# Autodesk Inventor assembly: Flap
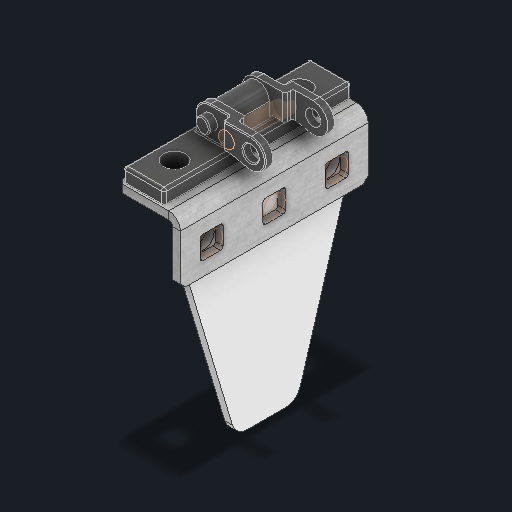
[picture p0: Inventor's stored thumbnail of the model, 512x512]
Saved by Autodesk Inventor 2025.1 (Build 291241000, 241)
## iProperties
Created: 2024-11-18
Part Number: Flap
Document SubType Name: Assembly
Designer: avere
Author: avere
## Documents named in this file (4)
- C:\Users\avere\VEX\High Stakes\CAD\V3\Intake\Floating Stage\Flap.iam
- C:\Users\avere\VEX\High Stakes\CAD\ROBOPROS-CAD-Inventor\Motion\Chain 9P\Chain Attachment Link.ipt
- C:\Users\avere\VEX\High Stakes\CAD\ROBOPROS-CAD-Inventor\Structure\Angle\Aluminum 1x1\Alu Angle 1x1x3.ipt
- C:\Users\avere\VEX\High Stakes\CAD\V3\Intake\Conveyer\Custom Parts\Hook Gusset.ipt
## Components (3 placed, 3 different names)
1. Chain Attachment Link:1 — Insert:3, Mate:3
2. Alu Angle 1x1x3:1 — Insert:2, Mate:2, Insert:3, Mate:3
3. Hook Gusset:1 — Insert:2, Mate:2
## Relationships (4: Insert 2, Mate 2)
- Insert:2: Alu Angle 1x1x3:1 ↔ Hook Gusset:1
- Mate:2: Alu Angle 1x1x3:1 ↔ Hook Gusset:1
- Insert:3: Chain Attachment Link:1 ↔ Alu Angle 1x1x3:1
- Mate:3: Chain Attachment Link:1 ↔ Alu Angle 1x1x3:1
